# Autodesk Inventor assembly: HOT-END
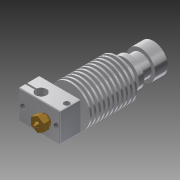
[picture p0: Inventor's stored thumbnail of the model, 180x180]
Saved by Autodesk Inventor 2014 SP1 (Build 180222100, 222)
## iProperties
Created: 2017-07-08
Part Number: HOT-END
Document SubType Name: Assembly
Designer: Stepan
Author: Stepan
## Documents named in this file (5)
- D:\3DPrinter\Hot-end\HOT-END.iam
- D:\3DPrinter\Hot-end\BLOCK-CARTRIDGE.ipt
- D:\3DPrinter\Hot-end\BREAK.ipt
- D:\3DPrinter\Hot-end\NOZZLE-ALL.ipt
- D:\3DPrinter\Hot-end\SINK-B.ipt
## Components (4 placed, 4 different names)
1. BLOCK-CARTRIDGE:1 — Жесткий:1, Вращательный:2
2. BREAK:1 — Вращательный:1, Жесткий:1
3. NOZZLE-ALL:1 — Вращательный:2
4. SINK-B:1 — Вращательный:1
## Relationships (3: RevoluteJoint 2, WeldJoint 1)
- Вращательный:1 [RevoluteJoint]: BREAK:1 ↔ SINK-B:1
- Жесткий:1 [WeldJoint]: BLOCK-CARTRIDGE:1 ↔ BREAK:1
- Вращательный:2 [RevoluteJoint]: BLOCK-CARTRIDGE:1 ↔ NOZZLE-ALL:1
